# Autodesk Inventor assembly: bearing
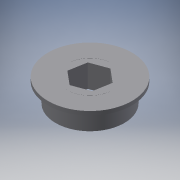
[picture p0: Inventor's stored thumbnail of the model, 180x180]
Saved by Autodesk Inventor 2017 (Build 210142000, 142)
## iProperties
Created: 2017-01-16
Part Number: bearing
Document SubType Name: Assembly
Designer: mmarkle
Author: mmarkle
## Documents named in this file (3)
- C:\Users\mmarkle\Documents\Robotics\Rope_Climber\bearing.iam
- C:\Users\mmarkle\Documents\Robotics\Rope_Climber\bearing_outer.ipt
- C:\Users\mmarkle\Documents\Robotics\Rope_Climber\bearing_inner.ipt
## Components (2 placed, 2 different names)
1. bearing_outer:1 — Insert:1
2. bearing_inner:1 — Insert:1
## Relationships (1: Insert 1)
- Insert:1: bearing_outer:1 ↔ bearing_inner:1
